# Autodesk Inventor assembly: 092_CPY1
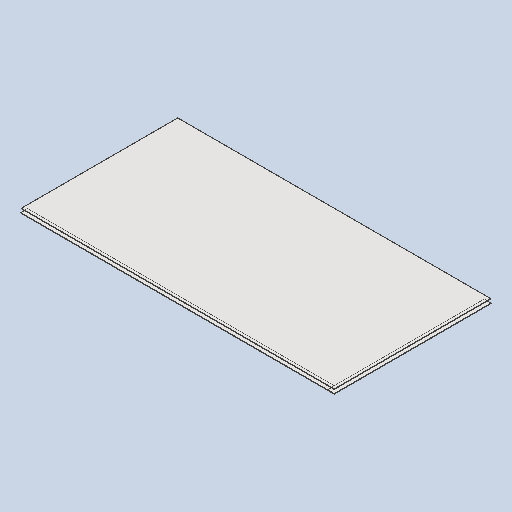
[picture p0: Inventor's stored thumbnail of the model, 512x512]
Saved by Autodesk Inventor 2026.2 (Build 302298000, 298)
## iProperties
Created: 2026-05-19
Part Number: 092_CPY1
Document SubType Name: Assembly
Designer: user
Author: user
## Documents named in this file (4)
- C:\Users\admin\Documents\Inventor\GBK-Gubkinskiy\092_CPY1.iam
- C:\Users\admin\Documents\Inventor\GBK-Gubkinskiy\0921_CPY1.ipt
- C:\Users\admin\Documents\Inventor\GBK-Gubkinskiy\0922_CPY1.ipt
- C:\Users\admin\Documents\Inventor\GBK-Gubkinskiy\0923_CPY1.ipt
## Components (3 placed, 3 different names)
1. 0921_CPY1:1 — Flush:1, Mate:1, Flush:2
2. 0922_CPY1:1 — Flush:1, Mate:1, Rigid:1
3. 0923_CPY1:1 — Flush:2, Rigid:1
## Relationships (4: Flush 2, Mate 1, WeldJoint 1)
- Flush:1 (34 mm): 0921_CPY1:1 ↔ 0922_CPY1:1
- Mate:1: 0921_CPY1:1 ↔ 0922_CPY1:1
- Flush:2 (34 mm): 0921_CPY1:1 ↔ 0923_CPY1:1
- Rigid:1 [WeldJoint]: 0922_CPY1:1 ↔ 0923_CPY1:1
